# Autodesk Inventor assembly: M178-REF-01
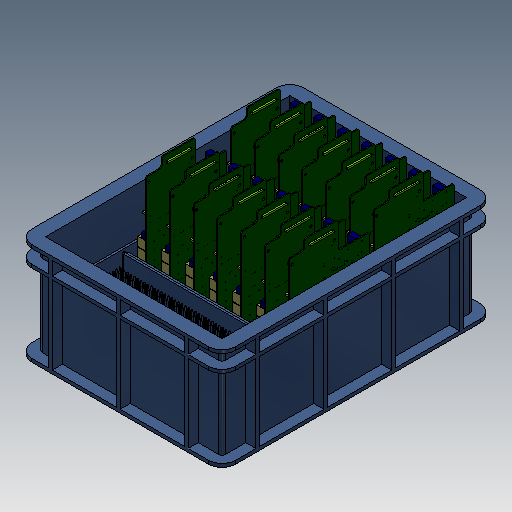
[picture p0: Inventor's stored thumbnail of the model, 512x512]
Saved by Autodesk Inventor 2018.3 (Build 223284000, 284)
## iProperties
Created: 2004-11-23
Document SubType Name: Assembly
Designer: Autodesk, Inc.
Manufacturer: Standard
Standards Organization: Custom
Part Number: M178-REF-01
Mass: 3534.78 g
Surface Area: 19733.6 cm^2
Volume: 3534.78 cm^3
Density: 1 g/cm^3
CAGE: 1LJX3
Dept. ID: Product Design
Description #2: ---
Finish #1: ---
Finish #2: ---
Material ID: ---
Project Number: ---
Author: Autodesk, Inc.
## Documents named in this file (4)
- C:\AVAInvAPI\Workspace\Test Station\Components\Filled Tote 2.iam
- C:\AVAInvAPI\Workspace\Test Station\Components\Standard Tote.iam
- C:\AVAInvAPI\Workspace\Test Station\Components\Slots Part 2.ipt
- C:\AVAInvAPI\Workspace\Test Station\Components\example2.max.ipt
## Components (19 placed, 3 different names)
1. Standard Tote:1 [sub-assembly] — Angle:2, Flush:1, Mate:1, Mate:2, Mate:3, Mate:4, Mate:6
2. Slots Part 2:1 — Angle:2, Flush:1, Mate:4, Mate:5, Flush:2
3. Slots Part 2:2 — Mate:5, Flush:2, Mate:6
4. Slots Part 2:3
5. Slots Part 2:4
6. example2.max:1 — Mate:1, Mate:2, Mate:3
7. example2.max:2
8. example2.max:3
9. example2.max:4
10. example2.max:5
11. example2.max:6
12. example2.max:7
13. example2.max:8
14. example2.max:9
15. example2.max:10
16. example2.max:11
17. example2.max:12
18. example2.max:13
19. example2.max:14
## Component patterns: (2 elements, first: Slots Part 2:1 + Slots Part 2:2), (14 elements, first: example2.max:1)
## Relationships (9: Mate 6, Flush 2, Angle 1)
- Angle:2 (0 deg): Standard Tote:1 ↔ Slots Part 2:1
- Flush:1: Standard Tote:1 ↔ Slots Part 2:1
- Mate:1: Standard Tote:1 ↔ example2.max:1
- Mate:2: Standard Tote:1 ↔ example2.max:1
- Mate:3: Standard Tote:1 ↔ example2.max:1
- Mate:4: Standard Tote:1 ↔ Slots Part 2:1
- Mate:5: Slots Part 2:1 ↔ Slots Part 2:2
- Flush:2: Slots Part 2:1 ↔ Slots Part 2:2
- Mate:6: Standard Tote:1 ↔ Slots Part 2:2
